# Autodesk Inventor assembly: standing_robot_ver.1
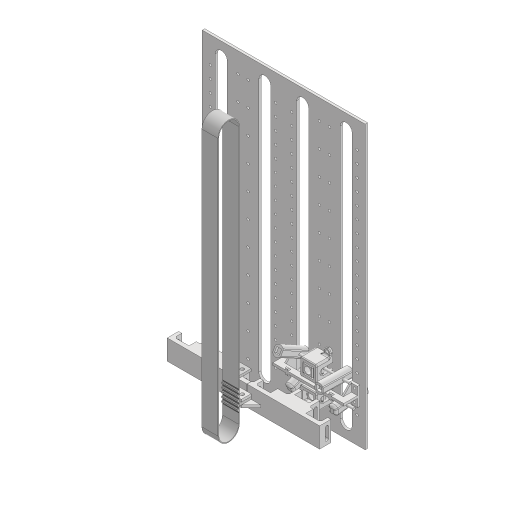
[picture p0: Inventor's stored thumbnail of the model, 512x512]
Saved by Autodesk Inventor 2024 (Build 280153000, 153)
## iProperties
Created: 2023-11-09
Part Number: standing_robot_ver.1
Document SubType Name: Assembly
Designer: moonshot
Author: moonshot
## Documents named in this file (9)
- C:\Users\moonshot\Desktop\ikisawa\ikisawa\experiment8_standing\standing_robot\standing_robot_ver.1.iam
- C:\Users\moonshot\Desktop\ikisawa\ikisawa\experiment8_standing\leg_unit\cover.ver1.ipt
- C:\Users\moonshot\Desktop\ikisawa\ikisawa\experiment8_standing\leg_unit\leg.ipt
- C:\Users\moonshot\Desktop\ikisawa\ikisawa\experiment8_standing\leg_unit\shaft_leg.ipt
- C:\Users\moonshot\Desktop\ikisawa\ikisawa\experiment8_standing\leg_unit\parent_ver.1.ipt
- C:\Users\moonshot\Desktop\ikisawa\ikisawa\experiment8_standing\floor\floor_ver.1.ipt
- C:\Users\moonshot\Desktop\ikisawa\ikisawa\experiment8_standing\belt\ATBT-720T5200-B-P30_info-1-16-16.ipt
- C:\Users\moonshot\Desktop\ikisawa\ikisawa\experiment8_standing\guide\guide_ver.2.ipt
- C:\Users\moonshot\Desktop\ikisawa\ikisawa\experiment8_standing\adapter\adapter_ver.1.ipt
## Components (15 placed, 8 different names)
1. cover.ver1:1 — フラッシュ:1, スライダ:1, メイト:8, メイト:9, メイト:10
2. leg:1 — メイト:2, メイト:5
3. leg:2 — メイト:3, メイト:4
4. shaft_leg:1 — メイト:1, フラッシュ:2, メイト:2, メイト:3
5. parent_ver.1:1 — フラッシュ:1, スライダ:1, メイト:1, フラッシュ:2
6. floor_ver.1:1 — フラッシュ:3, フラッシュ:4, フラッシュ:5, メイト:7, メイト:8, メイト:9, メイト:10, メイト:16, メイト:17, メイト:18, メイト:4, メイト:5, メイト:15, メイト:14, メイト:19, メイト:20, メイト:21
7. ATBT-720T5200-B-P30_info-1-16-16:1 — メイト:6, フラッシュ:6, メイト:7, メイト:22, メイト:23, メイト:24, メイト:25, メイト:26, メイト:27
8. cover.ver1:2 — メイト:16, メイト:17, メイト:18
9. leg:3 — メイト:15
10. leg:4 — メイト:14
11. shaft_leg:2
12. parent_ver.1:2
13. guide_ver.2:1 — メイト:19, メイト:20, メイト:21
14. adapter_ver.1:1 — メイト:22, メイト:23, メイト:24
15. adapter_ver.1:2 — メイト:25, メイト:26, メイト:27
## Relationships (37: Mate 27, Flush 8, TranslationJoint 2)
- フラッシュ:1 [Flush]: cover.ver1:1 ↔ parent_ver.1:1
- スライダ:1 [TranslationJoint]: cover.ver1:1 ↔ parent_ver.1:1
- メイト:1 [Mate]: shaft_leg:1 ↔ parent_ver.1:1
- フラッシュ:2 [Flush]: shaft_leg:1 ↔ parent_ver.1:1
- メイト:2 [Mate]: leg:1 ↔ shaft_leg:1
- メイト:3 [Mate]: leg:2 ↔ shaft_leg:1
- メイト:4 [Mate] (2.5 mm): leg:2 ↔ floor_ver.1:1
- メイト:5 [Mate] (2.5 mm): leg:1 ↔ floor_ver.1:1
- フラッシュ:3 [Flush]: floor_ver.1:1
- フラッシュ:4 [Flush]: floor_ver.1:1
- フラッシュ:5 [Flush]: floor_ver.1:1
- メイト:6 [Mate]: ATBT-720T5200-B-P30_info-1-16-16:1
- フラッシュ:6 [Flush]: ATBT-720T5200-B-P30_info-1-16-16:1
- メイト:7 [Mate] (50 mm): floor_ver.1:1 ↔ ATBT-720T5200-B-P30_info-1-16-16:1
- メイト:8 [Mate]: cover.ver1:1 ↔ floor_ver.1:1
- メイト:9 [Mate]: cover.ver1:1 ↔ floor_ver.1:1
- メイト:10 [Mate]: cover.ver1:1 ↔ floor_ver.1:1
- [Flush]: cover.ver1:2 ↔ parent_ver.1:2
- [TranslationJoint]: cover.ver1:2 ↔ parent_ver.1:2
- [Mate]: shaft_leg:2 ↔ parent_ver.1:2
- [Flush]: shaft_leg:2 ↔ parent_ver.1:2
- [Mate]: leg:3 ↔ shaft_leg:2
- [Mate]: leg:4 ↔ shaft_leg:2
- メイト:14 [Mate] (2.5 mm): floor_ver.1:1 ↔ leg:4
- メイト:15 [Mate] (2.5 mm): floor_ver.1:1 ↔ leg:3
- メイト:16 [Mate]: floor_ver.1:1 ↔ cover.ver1:2
- メイト:17 [Mate]: floor_ver.1:1 ↔ cover.ver1:2
- メイト:18 [Mate]: floor_ver.1:1 ↔ cover.ver1:2
- メイト:19 [Mate]: floor_ver.1:1 ↔ guide_ver.2:1
- メイト:20 [Mate]: floor_ver.1:1 ↔ guide_ver.2:1
- メイト:21 [Mate]: floor_ver.1:1 ↔ guide_ver.2:1
- メイト:22 [Mate]: ATBT-720T5200-B-P30_info-1-16-16:1 ↔ adapter_ver.1:1
- メイト:23 [Mate]: ATBT-720T5200-B-P30_info-1-16-16:1 ↔ adapter_ver.1:1
- メイト:24 [Mate]: ATBT-720T5200-B-P30_info-1-16-16:1 ↔ adapter_ver.1:1
- メイト:25 [Mate]: ATBT-720T5200-B-P30_info-1-16-16:1 ↔ adapter_ver.1:2
- メイト:26 [Mate]: ATBT-720T5200-B-P30_info-1-16-16:1 ↔ adapter_ver.1:2
- メイト:27 [Mate]: ATBT-720T5200-B-P30_info-1-16-16:1 ↔ adapter_ver.1:2
## Named parameters: d21_d1 = 0 mm, d22_d2 = 0 mm, d23_d3 = 2 mm, d24_d4 = -3 mm, d25_d5 = -3 mm, d26_d6 = 0 mm, d27_d7 = 0 mm, d28_d8 = 0 mm, d29_d9 = 0 mm, d30_d10 = 2.5 mm, d31_d11 = 2.5 mm
